# Autodesk Inventor assembly: koushika
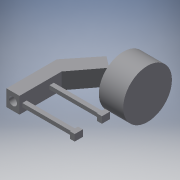
[picture p0: Inventor's stored thumbnail of the model, 180x180]
Saved by Autodesk Inventor 2019 (Build 230136000, 136)
## iProperties
Created: 2020-05-11
Part Number: koushika
Document SubType Name: Assembly
Designer: dvg
Author: dvg
## Documents named in this file (3)
- C:\Users\dvg\Documents\koushika.iam
- C:\Users\dvg\Documents\k.ipt
- C:\Users\dvg\Documents\k2.ipt
## Components (3 placed, 2 different names)
1. k:1 — Mate:1, Mate:2
2. k2:1 — Mate:1
3. k2:2 — Mate:2
## Relationships (2: Mate 2)
- Mate:1: k:1 ↔ k2:1
- Mate:2: k:1 ↔ k2:2
